# Autodesk Inventor assembly: SCHUNK-0331220 ERD 04-40-D-H-N, 0
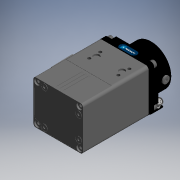
[picture p0: Inventor's stored thumbnail of the model, 180x180]
Saved by Autodesk Inventor 2017.3 (Build 213256000, 256)
## iProperties
Category: PARTsolutions
Company: SCHUNK
Part Number: SCHUNK-0331220 ERD 04-40-D-H-N, 0
Catalog Web Link: www.cadenas.de
Description: ERD-Rotary Units - Torque motor
Vendor: SCHUNK
Document SubType Name: Assembly
Designer: partserver
Manufacturer: SCHUNK
Mass: 1200 g
Surface Area: 699.923 cm^2
Volume: 491.545 cm^3
Density: 2.44128 g/cm^3
Title: SCHUNK-0331220 ERD 04-40-D-H-N
Author: Cadenas PARTsolutions
Comments: Rotary Units - Torque motor
PSOL_IDENT_0: {$CADENAS_DATA\23d-libs\schunk\greifsysteme\drehmodule\drehmodule_elektrisch\schwenkeinheiten\miniat
PSOL_IDENT_1: ur_schwenkeinheiten\erd_asm_at.prj},222 {VTYP=3D},{STYP=ASSTAB},{NB=SCHUNK-0331220 ERD 04-40-D-H-N,
PSOL_IDENT_2: 0},{LINA=SCHUNK-0331220 ERD 04-40-D-H-N},{NN=ERD},{DATE=23.04.2020 15:23:31},{GEOMDATE=15.04.2020 10
PSOL_IDENT_3: :30:43},{VERSION=},{LINEID=10},{WBVAR=SCWK},{WBNUMERIC=SCWK}  {NB=SCHUNK-0331220 ERD 04-40-D-H-N, 0
PSOL_IDENT_4: },{LINA=SCHUNK-0331220 ERD 04-40-D-H-N},{KT=DUMMY},{IDNR=0331220},{TYP=ERD 04-40-D-H-N},{ONLINE=Weit
PSOL_IDENT_5: ere Produktinformationen},{EPLAN=../../../../../produktbilder/icons/im0021678.png},{TYP1=1.000},{TYP
PSOL_IDENT_6: 2=1.000},{PPUE=8.000},{SCWK=0},{DDF=1.000},{IP=40.000},{TS=4.000},{FPLX=-23.500},{FPLY=74.000},{FPLZ=
PSOL_IDENT_7: 30.000},{NENNDREHMOMENT=0.400},{SPITZENDREHMOMEN=1.200},{MAXDREHZAHL=600},{MASSENTRAEGHEITS=500},{WI
PSOL_IDENT_8: EDERHOLGENAUIG=0.010},{FLUIDDURCHFUEHRU=2},{MAXBETRIEBSDRUCK=6},{EIGENMASSE=1.200},{UMGEBUNGSTEMPERA=
PSOL_IDENT_9: 10/40},{SCHUTZART=40},{SILZERTIFIZIERUN=nicht zertifiziert},{ZWISCHENKREISSPA=530},{NENNSTROM=0.430}
PSOL_IDENT_10: ,{MAXSTROM=1.290},{ANZAHLELEKTRODUR=4},{MAXSTROMEDF=1},{MAXSPANNUNGEDF=60},{POLPAARZAHL=7},{STEUEREL
PSOL_IDENT_11: EKTRONIK=extern},{GEBERSYSTEM=Encoder (absolut)},{AUSGANGSSIGNAL=Hiperface},{PPATH=erd_asmsbl.prj},{
PSOL_IDENT_12: PARTSERVER=1.000},{EPLANXX=https://eplandata.de/portal/portal.php?action=part-viewc&edpp=1.0&ev=1.9.
PSOL_IDENT_13: 11&lang=de_DE&clang=de_DE&mf=SNK&lastmpg=.&mcat=_eplan&tab=c&mcatsel=SNK},{EPLANXXX=https://eplandat
PSOL_IDENT_14: a.de/portal/portal.php?action=part-viewc&edpp=1.0&ev=1.9.11&lang=en_US&clang=en_US&lastmpg=.&tab=c&m
PSOL_IDENT_15: catsel=SNK},{EDZ=snk.0331220},{CNSCTN=85013100}
NB: SCHUNK-0331220 ERD 04-40-D-H-N, 0
NN: ERD
NT: Rotary Units - Torque motor
NBSYN: SCHUNK-$IDNR. $TYP., $SCWK.
LINA: SCHUNK-0331220 ERD 04-40-D-H-N
CATALOG: SCHUNK
IDNR: 0331220
TYP: ERD 04-40-D-H-N
ONLINE: Further product information
EPLAN: ../../../../../produktbilder/icons/im0021678.png
SCWK: 0
NENNDREHMOMENT: 0.4
SPITZENDREHMOMEN: 1.2
MAXDREHZAHL: 600
MASSENTRAEGHEITS: 500
WIEDERHOLGENAUIG: 0.01
FLUIDDURCHFUEHRU: 2
MAXBETRIEBSDRUCK: 6
EIGENMASSE: 1.2
UMGEBUNGSTEMPERA: 10/40
SCHUTZART: 40
SILZERTIFIZIERUN: not certified
ZWISCHENKREISSPA: 530
NENNSTROM: 0.43
MAXSTROM: 1.29
ANZAHLELEKTRODUR: 4
MAXSTROMEDF: 1
MAXSPANNUNGEDF: 60
POLPAARZAHL: 7
STEUERELEKTRONIK: external
GEBERSYSTEM: Encoder (absolute)
AUSGANGSSIGNAL: Hiperface
CNSCTN: 85013100
SUPPLIER: SCHUNK
ARTICLENO: SCHUNK-0331220 ERD 04-40-D-H-N, 0
BOMINFO: SCHUNK-0331220 ERD 04-40-D-H-N
CREATOR: CADENAS GmbH
## Documents named in this file (8)
- e:\temp\worker_34\temp\exporttempdir_1164_48_EsOKj\format_0\SCHUNK-0331220 ERD 04-40-D-H-N, 0.iam
- e:\temp\worker_34\temp\exporttempdir_1164_48_EsOKj\format_0\SCHUNK-0342382 Gehaeuse ERD 04.ipt
- e:\temp\worker_34\temp\exporttempdir_1164_48_EsOKj\format_0\SCHUNK-Deckel ERD.ipt
- e:\temp\worker_34\temp\exporttempdir_1164_48_EsOKj\format_0\Verschlussschraube DIN908 M7.ipt
- e:\temp\worker_34\temp\exporttempdir_1164_48_EsOKj\format_0\SCHUNK-Flansch IP 40 ERD.ipt
- e:\temp\worker_34\temp\exporttempdir_1164_48_EsOKj\format_0\SCHUNK-Stecker 2 ERD.ipt
- e:\temp\worker_34\temp\exporttempdir_1164_48_EsOKj\format_0\SCHUNK-9905502 Typenschild 9x24x0_3.ipt
- e:\temp\worker_34\temp\exporttempdir_1164_48_EsOKj\format_0\SCHUNK-Stecker ERD.ipt
## Components (10 placed, 7 different names)
1. SCHUNK-0342382 Gehaeuse ERD 04:1 — dec_XY@1 <-> geh_XY@2, dec_Z@1 <-> geh_Z@2, dec_YZ@1 <-> geh_YZ@2, stk_XY@1 <-> geh_XY@10, stk_Z@1 <-> geh_Z@10, stk_YZ@1 <-> geh_YZ@10
2. SCHUNK-Deckel ERD:1 — dec_XY@1 <-> geh_XY@2, dec_Z@1 <-> geh_Z@2, dec_YZ@1 <-> geh_YZ@2, vss2_XY@2 <-> din_908_XY@3, vss2_Z@2 <-> din_908_Z@3, vss2_YZ@2 <-> din_908_YZ@3, ring_XY@2 <-> ring_stk_XY@4, ring_Z@2 <-> ring_stk_Z@4, ring_YZ@2 <-> ring_stk_YZ@4, vss1_XY@2 <-> din_908_XY@8, vss1_Z@2 <-> din_908_Z@8, vss1_YZ@2 <-> din_908_YZ@8, typenschild_XY@2 <-> aluschild_XY@9, typenschild_Z@2 <-> aluschild_Z@9, typenschild_YZ@2 <-> aluschild_YZ@9
3. Verschlussschraube DIN908 M7:1 — vss2_XY@2 <-> din_908_XY@3, vss2_Z@2 <-> din_908_Z@3, vss2_YZ@2 <-> din_908_YZ@3
4. SCHUNK-Flansch IP 40 ERD:1 — ring_XY@2 <-> ring_stk_XY@4, ring_Z@2 <-> ring_stk_Z@4, ring_YZ@2 <-> ring_stk_YZ@4, vss1_XY@4 <-> din_908_XY@5, vss1_Z@4 <-> din_908_Z@5, vss1_YZ@4 <-> din_908_YZ@5, vss2_XY@4 <-> din_908_XY@6, vss2_Z@4 <-> din_908_Z@6, vss2_YZ@4 <-> din_908_YZ@6, stecker_XY@4 <-> welle_XY@7, stecker_Z@4 <-> welle_Z@7, stecker_YZ@4 <-> welle_YZ@7
5. Verschlussschraube DIN908 M7:2 — vss1_XY@4 <-> din_908_XY@5, vss1_Z@4 <-> din_908_Z@5, vss1_YZ@4 <-> din_908_YZ@5
6. Verschlussschraube DIN908 M7:3 — vss2_XY@4 <-> din_908_XY@6, vss2_Z@4 <-> din_908_Z@6, vss2_YZ@4 <-> din_908_YZ@6
7. SCHUNK-Stecker 2 ERD:1 — stecker_XY@4 <-> welle_XY@7, stecker_Z@4 <-> welle_Z@7, stecker_YZ@4 <-> welle_YZ@7
8. Verschlussschraube DIN908 M7:4 — vss1_XY@2 <-> din_908_XY@8, vss1_Z@2 <-> din_908_Z@8, vss1_YZ@2 <-> din_908_YZ@8
9. SCHUNK-9905502 Typenschild 9x24x0_3:1 — typenschild_XY@2 <-> aluschild_XY@9, typenschild_Z@2 <-> aluschild_Z@9, typenschild_YZ@2 <-> aluschild_YZ@9
10. SCHUNK-Stecker ERD:1 — stk_XY@1 <-> geh_XY@10, stk_Z@1 <-> geh_Z@10, stk_YZ@1 <-> geh_YZ@10
## Relationships (27: Mate 10, Angle 9, Flush 8)
- dec_XY@1 <-> geh_XY@2 [Flush]: SCHUNK-0342382 Gehaeuse ERD 04:1 ↔ SCHUNK-Deckel ERD:1
- dec_Z@1 <-> geh_Z@2 [Mate]: SCHUNK-0342382 Gehaeuse ERD 04:1 ↔ SCHUNK-Deckel ERD:1
- dec_YZ@1 <-> geh_YZ@2 [Angle] (90 deg): SCHUNK-0342382 Gehaeuse ERD 04:1 ↔ SCHUNK-Deckel ERD:1
- vss2_XY@2 <-> din_908_XY@3 [Flush]: SCHUNK-Deckel ERD:1 ↔ Verschlussschraube DIN908 M7:1
- vss2_Z@2 <-> din_908_Z@3 [Mate]: SCHUNK-Deckel ERD:1 ↔ Verschlussschraube DIN908 M7:1
- vss2_YZ@2 <-> din_908_YZ@3 [Angle] (0 deg): SCHUNK-Deckel ERD:1 ↔ Verschlussschraube DIN908 M7:1
- ring_XY@2 <-> ring_stk_XY@4 [Flush]: SCHUNK-Deckel ERD:1 ↔ SCHUNK-Flansch IP 40 ERD:1
- ring_Z@2 <-> ring_stk_Z@4 [Mate]: SCHUNK-Deckel ERD:1 ↔ SCHUNK-Flansch IP 40 ERD:1
- ring_YZ@2 <-> ring_stk_YZ@4 [Angle] (180 deg): SCHUNK-Deckel ERD:1 ↔ SCHUNK-Flansch IP 40 ERD:1
- vss1_XY@4 <-> din_908_XY@5 [Flush]: SCHUNK-Flansch IP 40 ERD:1 ↔ Verschlussschraube DIN908 M7:2
- vss1_Z@4 <-> din_908_Z@5 [Mate]: SCHUNK-Flansch IP 40 ERD:1 ↔ Verschlussschraube DIN908 M7:2
- vss1_YZ@4 <-> din_908_YZ@5 [Angle] (0 deg): SCHUNK-Flansch IP 40 ERD:1 ↔ Verschlussschraube DIN908 M7:2
- vss2_XY@4 <-> din_908_XY@6 [Flush]: SCHUNK-Flansch IP 40 ERD:1 ↔ Verschlussschraube DIN908 M7:3
- vss2_Z@4 <-> din_908_Z@6 [Mate]: SCHUNK-Flansch IP 40 ERD:1 ↔ Verschlussschraube DIN908 M7:3
- vss2_YZ@4 <-> din_908_YZ@6 [Angle] (0 deg): SCHUNK-Flansch IP 40 ERD:1 ↔ Verschlussschraube DIN908 M7:3
- stecker_XY@4 <-> welle_XY@7 [Flush]: SCHUNK-Flansch IP 40 ERD:1 ↔ SCHUNK-Stecker 2 ERD:1
- stecker_Z@4 <-> welle_Z@7 [Mate]: SCHUNK-Flansch IP 40 ERD:1 ↔ SCHUNK-Stecker 2 ERD:1
- stecker_YZ@4 <-> welle_YZ@7 [Angle] (-4.5 deg): SCHUNK-Flansch IP 40 ERD:1 ↔ SCHUNK-Stecker 2 ERD:1
- vss1_XY@2 <-> din_908_XY@8 [Flush]: SCHUNK-Deckel ERD:1 ↔ Verschlussschraube DIN908 M7:4
- vss1_Z@2 <-> din_908_Z@8 [Mate]: SCHUNK-Deckel ERD:1 ↔ Verschlussschraube DIN908 M7:4
- vss1_YZ@2 <-> din_908_YZ@8 [Angle] (0 deg): SCHUNK-Deckel ERD:1 ↔ Verschlussschraube DIN908 M7:4
- typenschild_XY@2 <-> aluschild_XY@9 [Flush]: SCHUNK-Deckel ERD:1 ↔ SCHUNK-9905502 Typenschild 9x24x0_3:1
- typenschild_Z@2 <-> aluschild_Z@9 [Mate]: SCHUNK-Deckel ERD:1 ↔ SCHUNK-9905502 Typenschild 9x24x0_3:1
- typenschild_YZ@2 <-> aluschild_YZ@9 [Angle] (180 deg): SCHUNK-Deckel ERD:1 ↔ SCHUNK-9905502 Typenschild 9x24x0_3:1
- stk_XY@1 <-> geh_XY@10 [Mate]: SCHUNK-0342382 Gehaeuse ERD 04:1 ↔ SCHUNK-Stecker ERD:1
- stk_Z@1 <-> geh_Z@10 [Mate]: SCHUNK-0342382 Gehaeuse ERD 04:1 ↔ SCHUNK-Stecker ERD:1
- stk_YZ@1 <-> geh_YZ@10 [Angle] (-90 deg): SCHUNK-0342382 Gehaeuse ERD 04:1 ↔ SCHUNK-Stecker ERD:1
